# Autodesk Inventor assembly: Assemlby_TIRFImager_50mmNEMA_v3
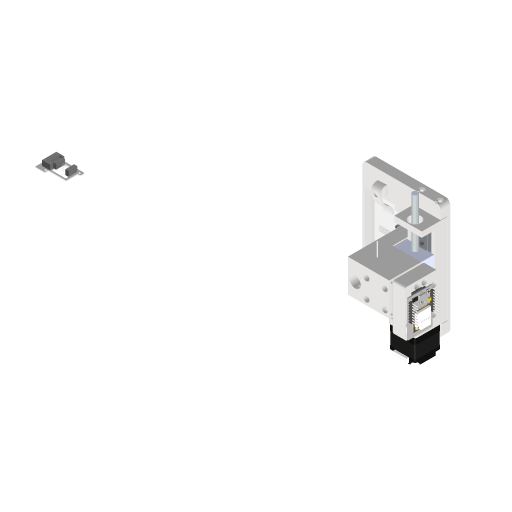
[picture p0: Inventor's stored thumbnail of the model, 512x512]
Saved by Autodesk Inventor 2024.1 (Build 281209000, 209)
## iProperties
Created: 2022-05-21
Part Number: Assemlby_TIRFImager_50mmNEMA_v3
Document SubType Name: Assembly
Designer: diederichbenedict
Author: diederichbenedict
## Documents named in this file (14)
- C:\Users\diederichbenedict\Dropbox\Dokumente\Promotion\PROJECTS\TIRFImager\INVENTOR\Assemlby_TIRFImager_50mmNEMA_v3.iam
- C:\Users\diederichbenedict\Dropbox\Dokumente\Promotion\PROJECTS\TIRFImager\INVENTOR\00_chipnano_waveguide_slidsize.ipt
- C:\Users\diederichbenedict\Dropbox\Dokumente\Promotion\PROJECTS\TIRFImager\INVENTOR\00_KES400.iam
- C:\Users\diederichbenedict\Dropbox\Dokumente\Promotion\PROJECTS\TIRFImager\INVENTOR\30_XYTabel_Aliexpress_cellSTORM_chiptray_clamp.ipt
- C:\Users\diederichbenedict\Dropbox\Dokumente\Promotion\PROJECTS\TIRFImager\INVENTOR\30_XYTabel_Aliexpress_cellSTORM_chiptray_spacer.ipt
- C:\Users\diederichbenedict\Dropbox\Dokumente\Promotion\PROJECTS\TIRFImager\INVENTOR\00_Linear_Stage_NEMA11_china.iam
- C:\Users\diederichbenedict\Dropbox\Dokumente\Promotion\PROJECTS\TIRFImager\INVENTOR\00_Carriage.ipt
- C:\Users\diederichbenedict\Dropbox\Dokumente\Promotion\PROJECTS\TIRFImager\INVENTOR\00_Comar_Mirror.ipt
- C:\Users\diederichbenedict\Dropbox\Dokumente\Promotion\PROJECTS\TIRFImager\INVENTOR\ESP3-CAM v4.iam
- C:\Users\diederichbenedict\Dropbox\Dokumente\Promotion\PROJECTS\TIRFImager\INVENTOR\00_cctvlens.ipt
- C:\Users\diederichbenedict\Dropbox\Dokumente\Promotion\PROJECTS\TIRFImager\INVENTOR\30_ESP32_Camera_tray.ipt
- C:\Users\diederichbenedict\Dropbox\Dokumente\Promotion\PROJECTS\TIRFImager\INVENTOR\30_Cameraholder.ipt
- C:\Users\diederichbenedict\Dropbox\Dokumente\Promotion\PROJECTS\TIRFImager\INVENTOR\TIRFImager_base_50mm_NEMA11_v3.ipt
- C:\Users\diederichbenedict\Dropbox\Dokumente\Promotion\PROJECTS\TIRFImager\INVENTOR\TIRFImager_Laserbase_v3.ipt
## Components (15 placed, 13 different names)
1. TIRFImager_base_50mm_NEMA11_v3:1 — Passend:1, Fluchtend:1, Fluchtend:2, Einfügen:1, Einfügen:2, Fluchtend:8, Fluchtend:9, Fluchtend:10, Fluchtend:11, Fluchtend:12, Winkel:6, Winkel:7, Winkel:8
2. 00_chipnano_waveguide_slidsize:1 — Passend:1, Fluchtend:1, Fluchtend:2, Passend:13
3. 30_XYTabel_Aliexpress_cellSTORM_chiptray_clamp:1 — Einfügen:1
4. 30_XYTabel_Aliexpress_cellSTORM_chiptray_clamp:2 — Einfügen:2
5. 30_XYTabel_Aliexpress_cellSTORM_chiptray_spacer:1
6. 00_Carriage:1 — Passend:12, Winkel:5, Fluchtend:13, Fluchtend:14
7. 00_Comar_Mirror:1
8. 00_cctvlens:1 — Passend:10
9. ESP3-CAM v4:1 [sub-assembly] — Passend:10, Winkel:4, Passend:11
10. 30_ESP32_Camera_tray:1 — Winkel:4, Passend:11
11. 30_Cameraholder:1 — Fluchtend:8, Fluchtend:9
12. 00_Linear_Stage_NEMA11_china:1 [sub-assembly] — Fluchtend:10, Fluchtend:11, Fluchtend:12, Passend:12, Winkel:5
13. 00_KES400:2 [sub-assembly]
14. 00_KES400:3 [sub-assembly] — Passend:13, Winkel:6, Einfügen:3
15. TIRFImager_Laserbase_v3:1 — Einfügen:3, Winkel:7, Winkel:8, Fluchtend:13, Fluchtend:14
## Relationships (22: Flush 9, Mate 5, Angle 5, Insert 3)
- Passend:1 [Mate]: TIRFImager_base_50mm_NEMA11_v3:1 ↔ 00_chipnano_waveguide_slidsize:1
- Fluchtend:1 [Flush] (1 mm): TIRFImager_base_50mm_NEMA11_v3:1 ↔ 00_chipnano_waveguide_slidsize:1
- Fluchtend:2 [Flush] (4 mm): TIRFImager_base_50mm_NEMA11_v3:1 ↔ 00_chipnano_waveguide_slidsize:1
- Einfügen:1 [Insert]: TIRFImager_base_50mm_NEMA11_v3:1 ↔ 30_XYTabel_Aliexpress_cellSTORM_chiptray_clamp:1
- Einfügen:2 [Insert]: TIRFImager_base_50mm_NEMA11_v3:1 ↔ 30_XYTabel_Aliexpress_cellSTORM_chiptray_clamp:2
- Passend:10 [Mate]: 00_cctvlens:1 ↔ ESP3-CAM v4:1
- Winkel:4 [Angle] (0 deg): ESP3-CAM v4:1 ↔ 30_ESP32_Camera_tray:1
- Passend:11 [Mate] (12 mm): ESP3-CAM v4:1 ↔ 30_ESP32_Camera_tray:1
- Fluchtend:8 [Flush]: TIRFImager_base_50mm_NEMA11_v3:1 ↔ 30_Cameraholder:1
- Fluchtend:9 [Flush]: TIRFImager_base_50mm_NEMA11_v3:1 ↔ 30_Cameraholder:1
- Fluchtend:10 [Flush]: TIRFImager_base_50mm_NEMA11_v3:1 ↔ 00_Linear_Stage_NEMA11_china:1
- Fluchtend:11 [Flush] (15 mm): TIRFImager_base_50mm_NEMA11_v3:1 ↔ 00_Linear_Stage_NEMA11_china:1
- Fluchtend:12 [Flush] (3 mm): TIRFImager_base_50mm_NEMA11_v3:1 ↔ 00_Linear_Stage_NEMA11_china:1
- Passend:12 [Mate]: 00_Carriage:1 ↔ 00_Linear_Stage_NEMA11_china:1
- Winkel:5 [Angle] (180 deg): 00_Carriage:1 ↔ 00_Linear_Stage_NEMA11_china:1
- Passend:13 [Mate]: 00_chipnano_waveguide_slidsize:1 ↔ 00_KES400:3
- Winkel:6 [Angle] (0 deg): TIRFImager_base_50mm_NEMA11_v3:1 ↔ 00_KES400:3
- Einfügen:3 [Insert]: 00_KES400:3 ↔ TIRFImager_Laserbase_v3:1
- Winkel:7 [Angle] (90 deg): TIRFImager_base_50mm_NEMA11_v3:1 ↔ TIRFImager_Laserbase_v3:1
- Winkel:8 [Angle] (180 deg): TIRFImager_base_50mm_NEMA11_v3:1 ↔ TIRFImager_Laserbase_v3:1
- Fluchtend:13 [Flush]: 00_Carriage:1 ↔ TIRFImager_Laserbase_v3:1
- Fluchtend:14 [Flush]: 00_Carriage:1 ↔ TIRFImager_Laserbase_v3:1
